# Autodesk Inventor assembly: Drive Roller Assembly
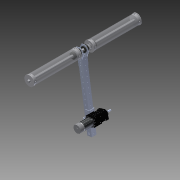
[picture p0: Inventor's stored thumbnail of the model, 180x180]
Saved by Autodesk Inventor 2014 (Build 180170000, 170)
## iProperties
Created: 2014-01-12
Part Number: Drive Roller Assembly
Document SubType Name: Assembly
Designer: Michael
Mass: 1125.53 g
Surface Area: 3756.72 cm^2
Volume: 516.176 cm^3
Density: 2.18052 g/cm^3
Author: Michael
## Documents named in this file (17)
- C:\Users\Michael\Documents\GitHub\2014buildCAD\Collector\Drive Roller Assembly.iam
- C:\Users\Michael\Documents\GitHub\2014buildCAD\Collector\Hex Shaft Collar 1-2 in (7552K500).ipt
- C:\Users\Michael\Documents\GitHub\2014buildCAD\Collector\Timing Pulley (HTD 5mm) - 18T 9mm Double Flange, 1-2 in Hex (VexPro).ipt
- C:\Users\Michael\Documents\GitHub\2014buildCAD\Collector\Hex Bearing 1-2 in (FR8ZZ-Hex, am-0279).ipt
- C:\Users\Michael\Documents\GitHub\2014buildCAD\Collector\Roller End Cap Drive (3-D Printed).ipt
- C:\Users\Michael\Documents\GitHub\2014buildCAD\Funnel Catcher\Vex Pro End Bearing Mount.ipt
- C:\Users\Michael\Documents\GitHub\2014buildCAD\Funnel Catcher\Vex Pro 1x1 rectangular tubing 14 in length.ipt
- C:\Users\Michael\Documents\GitHub\2014buildCAD\Collector\VersaPlanetary.iam
- C:\Users\Michael\Documents\GitHub\2014buildCAD\Collector\Vex Pro VersaPlanetary Side Mount.ipt
- C:\Users\Michael\Documents\GitHub\2014buildCAD\Collector\Polycarbonate Roller 2 OD 1-16 Thick (8585K64).ipt
- C:\Users\Michael\Documents\GitHub\2014buildCAD\Collector\Hex Shaft Aluminum 1-2 in (am-2291).ipt
- C:\Users\Arpan\Documents\GitHub\2014buildCAD\Collector\Drive Roller Assembly\AIP\FEA\axi0epmtc.fins
- C:\Users\Arpan\Documents\GitHub\2014buildCAD\Collector\Drive Roller Assembly\AIP\FEA\axi0epmu8.fsat
- C:\Users\Arpan\Documents\GitHub\2014buildCAD\Collector\Drive Roller Assembly\AIP\FEA\axi0epmu8.ftes
- C:\Users\Arpan\Documents\GitHub\2014buildCAD\Collector\Drive Roller Assembly\AIP\FEA\axi0epmu8.fwiz
- C:\Users\Arpan\Documents\GitHub\2014buildCAD\Collector\Drive Roller Assembly\AIP\FEA\axi0epnk0.fmsh
- C:\Users\Arpan\Documents\GitHub\2014buildCAD\Collector\Drive Roller Assembly\AIP\FEA\axi0epoao.fres
## Components (19 placed, 10 different names)
1. Timing Pulley (HTD 5mm) - 18T 9mm Double Flange, 1-2 in Hex (VexPro):1 — Mate:49, Mate:50, Mate:107, Mate:108
2. Hex Bearing 1-2 in (FR8ZZ-Hex, am-0279):1 — Insert:8, Mate:55, Mate:96, Mate:97
3. Hex Shaft Collar 1-2 in (7552K500):5 — Mate:50, Mate:55, Mate:105, Mate:106
4. Roller End Cap Drive (3-D Printed):1 — Mate:49, Insert:25, Mate:86, Mate:90, Mate:111, Mate:112
5. Vex Pro End Bearing Mount:1 — Insert:8, Mate:58, Insert:15, Insert:16
6. Hex Bearing 1-2 in (FR8ZZ-Hex, am-0279):2 — Insert:9, Mate:61, Mate:98
7. Hex Shaft Collar 1-2 in (7552K500):6 — Mate:61, Mate:83, Mate:99, Mate:100
8. Vex Pro End Bearing Mount:2 — Mate:58, Insert:9, Insert:13, Insert:14
9. Roller End Cap Drive (3-D Printed):2 — Insert:26, Mate:95, Flush:1
10. Vex Pro 1x1 rectangular tubing 14 in length:1 — Insert:13, Insert:14, Insert:15, Insert:16, Insert:23, Insert:24
11. VersaPlanetary:1 [sub-assembly] — Insert:21, Insert:22
12. Vex Pro VersaPlanetary Side Mount:1 — Insert:21, Insert:22, Insert:23, Insert:24
13. Roller End Cap Drive (3-D Printed):3 — Mate:83, Mate:87, Insert:28, Mate:93, Mate:103, Mate:104
14. Polycarbonate Roller 2 OD 1-16 Thick (8585K64):1 — Insert:25, Mate:86, Insert:26, Rotation:1, Mate:95
15. Roller End Cap Drive (3-D Printed):4 — Mate:94
16. Polycarbonate Roller 2 OD 1-16 Thick (8585K64):2 — Insert:28, Mate:93, Mate:94, Rotation:1
17. Hex Shaft Collar 1-2 in (7552K500):7 — Mate:87, Mate:101, Mate:102
18. Hex Shaft Collar 1-2 in (7552K500):8 — Mate:90, Mate:109, Mate:110
19. Hex Shaft Aluminum 1-2 in (am-2291):1 — Mate:96, Mate:97, Mate:98, Mate:99, Mate:100, Mate:101, Mate:102, Mate:103, Mate:104, Mate:105, Mate:106, Mate:107, Mate:108, Mate:109, Mate:110, Mate:111, Mate:112, Flush:1
## Relationships (45: Mate 29, Insert 14, RelateRotation 1, Flush 1)
- Mate:49: Timing Pulley (HTD 5mm) - 18T 9mm Double Flange, 1-2 in Hex (VexPro):1 ↔ Roller End Cap Drive (3-D Printed):1
- Mate:50: Timing Pulley (HTD 5mm) - 18T 9mm Double Flange, 1-2 in Hex (VexPro):1 ↔ Hex Shaft Collar 1-2 in (7552K500):5
- Insert:8: Hex Bearing 1-2 in (FR8ZZ-Hex, am-0279):1 ↔ Vex Pro End Bearing Mount:1
- Mate:55: Hex Bearing 1-2 in (FR8ZZ-Hex, am-0279):1 ↔ Hex Shaft Collar 1-2 in (7552K500):5
- Mate:58 (25.4 mm): Vex Pro End Bearing Mount:1 ↔ Vex Pro End Bearing Mount:2
- Insert:9: Hex Bearing 1-2 in (FR8ZZ-Hex, am-0279):2 ↔ Vex Pro End Bearing Mount:2
- Mate:61: Hex Bearing 1-2 in (FR8ZZ-Hex, am-0279):2 ↔ Hex Shaft Collar 1-2 in (7552K500):6
- Insert:13: Vex Pro End Bearing Mount:2 ↔ Vex Pro 1x1 rectangular tubing 14 in length:1
- Insert:14: Vex Pro End Bearing Mount:2 ↔ Vex Pro 1x1 rectangular tubing 14 in length:1
- Insert:15: Vex Pro End Bearing Mount:1 ↔ Vex Pro 1x1 rectangular tubing 14 in length:1
- Insert:16: Vex Pro End Bearing Mount:1 ↔ Vex Pro 1x1 rectangular tubing 14 in length:1
- Insert:21: VersaPlanetary:1 ↔ Vex Pro VersaPlanetary Side Mount:1
- Insert:22: VersaPlanetary:1 ↔ Vex Pro VersaPlanetary Side Mount:1
- Insert:23: Vex Pro 1x1 rectangular tubing 14 in length:1 ↔ Vex Pro VersaPlanetary Side Mount:1
- Insert:24: Vex Pro 1x1 rectangular tubing 14 in length:1 ↔ Vex Pro VersaPlanetary Side Mount:1
- Mate:83: Hex Shaft Collar 1-2 in (7552K500):6 ↔ Roller End Cap Drive (3-D Printed):3
- Insert:25: Roller End Cap Drive (3-D Printed):1 ↔ Polycarbonate Roller 2 OD 1-16 Thick (8585K64):1
- Mate:86: Roller End Cap Drive (3-D Printed):1 ↔ Polycarbonate Roller 2 OD 1-16 Thick (8585K64):1
- Insert:26: Roller End Cap Drive (3-D Printed):2 ↔ Polycarbonate Roller 2 OD 1-16 Thick (8585K64):1
- [Insert]: Roller End Cap Drive (3-D Printed):4 ↔ Polycarbonate Roller 2 OD 1-16 Thick (8585K64):2
- Mate:87: Roller End Cap Drive (3-D Printed):3 ↔ Hex Shaft Collar 1-2 in (7552K500):7
- Mate:90: Roller End Cap Drive (3-D Printed):1 ↔ Hex Shaft Collar 1-2 in (7552K500):8
- Insert:28: Roller End Cap Drive (3-D Printed):3 ↔ Polycarbonate Roller 2 OD 1-16 Thick (8585K64):2
- Mate:93: Roller End Cap Drive (3-D Printed):3 ↔ Polycarbonate Roller 2 OD 1-16 Thick (8585K64):2
- Mate:94: Roller End Cap Drive (3-D Printed):4 ↔ Polycarbonate Roller 2 OD 1-16 Thick (8585K64):2
- Rotation:1 [RelateRotation] (1 ul): Polycarbonate Roller 2 OD 1-16 Thick (8585K64):1 ↔ Polycarbonate Roller 2 OD 1-16 Thick (8585K64):2
- Mate:95: Roller End Cap Drive (3-D Printed):2 ↔ Polycarbonate Roller 2 OD 1-16 Thick (8585K64):1
- Mate:96: Hex Bearing 1-2 in (FR8ZZ-Hex, am-0279):1 ↔ Hex Shaft Aluminum 1-2 in (am-2291):1
- Mate:97: Hex Bearing 1-2 in (FR8ZZ-Hex, am-0279):1 ↔ Hex Shaft Aluminum 1-2 in (am-2291):1
- Mate:98: Hex Bearing 1-2 in (FR8ZZ-Hex, am-0279):2 ↔ Hex Shaft Aluminum 1-2 in (am-2291):1
- Mate:99: Hex Shaft Collar 1-2 in (7552K500):6 ↔ Hex Shaft Aluminum 1-2 in (am-2291):1
- Mate:100: Hex Shaft Collar 1-2 in (7552K500):6 ↔ Hex Shaft Aluminum 1-2 in (am-2291):1
- Mate:101: Hex Shaft Collar 1-2 in (7552K500):7 ↔ Hex Shaft Aluminum 1-2 in (am-2291):1
- Mate:102: Hex Shaft Collar 1-2 in (7552K500):7 ↔ Hex Shaft Aluminum 1-2 in (am-2291):1
- Mate:103: Roller End Cap Drive (3-D Printed):3 ↔ Hex Shaft Aluminum 1-2 in (am-2291):1
- Mate:104: Roller End Cap Drive (3-D Printed):3 ↔ Hex Shaft Aluminum 1-2 in (am-2291):1
- Mate:105: Hex Shaft Collar 1-2 in (7552K500):5 ↔ Hex Shaft Aluminum 1-2 in (am-2291):1
- Mate:106: Hex Shaft Collar 1-2 in (7552K500):5 ↔ Hex Shaft Aluminum 1-2 in (am-2291):1
- Mate:107: Timing Pulley (HTD 5mm) - 18T 9mm Double Flange, 1-2 in Hex (VexPro):1 ↔ Hex Shaft Aluminum 1-2 in (am-2291):1
- Mate:108: Timing Pulley (HTD 5mm) - 18T 9mm Double Flange, 1-2 in Hex (VexPro):1 ↔ Hex Shaft Aluminum 1-2 in (am-2291):1
- Mate:109: Hex Shaft Collar 1-2 in (7552K500):8 ↔ Hex Shaft Aluminum 1-2 in (am-2291):1
- Mate:110: Hex Shaft Collar 1-2 in (7552K500):8 ↔ Hex Shaft Aluminum 1-2 in (am-2291):1
- Mate:111: Roller End Cap Drive (3-D Printed):1 ↔ Hex Shaft Aluminum 1-2 in (am-2291):1
- Mate:112: Roller End Cap Drive (3-D Printed):1 ↔ Hex Shaft Aluminum 1-2 in (am-2291):1
- Flush:1 (-9.525 mm): Roller End Cap Drive (3-D Printed):2 ↔ Hex Shaft Aluminum 1-2 in (am-2291):1
## Named parameters: sa_0 = -444.138, sa_1 = 24.6654, sa_2 = 0, d138_d137 = 0 mm, sa_3 = 8896.44
note: some values were not read from the file. Shown as the stored number, unit unknown: "sa_0", "sa_1", "sa_2", "sa_3".
